# Autodesk Inventor assembly: Assembly1
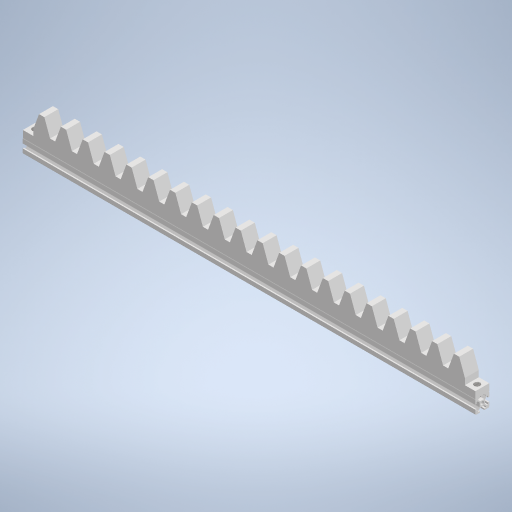
[picture p0: Inventor's stored thumbnail of the model, 512x512]
Saved by Autodesk Inventor 2023.2 (Build 272271030, 271C)
## iProperties
Created: 2023-03-04
Part Number: Assembly1
Document SubType Name: Assembly
Designer: Cris Pat
Author: Cris Pat
## Documents named in this file (5)
- C:\Users\Cris Pat\Desktop\U\Semestre 9\disenio e innovacion\CAD\Hbot\eje.iam
- C:\Users\Cris Pat\Desktop\U\Semestre 9\disenio e innovacion\CAD\Hbot\cremallera1.ipt
- C:\Users\Cris Pat\Desktop\U\Semestre 9\disenio e innovacion\CAD\Hbot\perfil_2020T.ipt
- C:\Users\Cris Pat\Desktop\U\Semestre 9\disenio e innovacion\CAD\Hbot\libreria\en-US\DIN 84\DIN 84 - M5 x 12.ipt
- C:\Users\Cris Pat\Desktop\U\Semestre 9\disenio e innovacion\CAD\Hbot\libreria\en-US\DIN 439-2\DIN 439 - M5 x 0.8.ipt
## Components (6 placed, 4 different names)
1. cremallera1:1 — Flush:3, Flush:4, Flush:5, Mate:3, Insert:1, Insert:2
2. perfil_2020T:1 — Flush:4, Flush:5, Mate:3
3. DIN 84 - replaced by DIN EN ISO 1207 M5 x 12:1 — Insert:1, Mate:5
4. DIN 84 - replaced by DIN EN ISO 1207 M5 x 12:2 — Insert:2, Mate:4
5. DIN 439-2 - replaced by DIN EN 24035/28675 M5:1 — Mate:4
6. DIN 439-2 - replaced by DIN EN 24035/28675 M5:2 — Mate:5
## Relationships (9: Flush 4, Mate 3, Insert 2)
- Flush:2 (-100 mm)
- Flush:3 (12.5 mm): cremallera1:1
- Flush:4: cremallera1:1 ↔ perfil_2020T:1
- Flush:5: cremallera1:1 ↔ perfil_2020T:1
- Mate:3: cremallera1:1 ↔ perfil_2020T:1
- Insert:1: cremallera1:1 ↔ DIN 84 - replaced by DIN EN ISO 1207 M5 x 12:1
- Insert:2: cremallera1:1 ↔ DIN 84 - replaced by DIN EN ISO 1207 M5 x 12:2
- Mate:4: DIN 84 - replaced by DIN EN ISO 1207 M5 x 12:2 ↔ DIN 439-2 - replaced by DIN EN 24035/28675 M5:1
- Mate:5: DIN 84 - replaced by DIN EN ISO 1207 M5 x 12:1 ↔ DIN 439-2 - replaced by DIN EN 24035/28675 M5:2
